# Autodesk Inventor assembly: 17-0028-0121
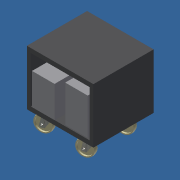
[picture p0: Inventor's stored thumbnail of the model, 180x180]
Saved by Autodesk Inventor 2019.1 (Build 231200000, 200)
## iProperties
Created: 2018-12-19
Part Number: 17-0028-0121
Document SubType Name: Assembly
Designer: D. Giesen
Author: D. Giesen
## Documents named in this file (4)
- D:\VaultLocalWorkingFolder\UvA_MT\Projects\2017\17-0028 Digital PID Loop\10_Assemblies\17-0028-0121.iam
- D:\VaultLocalWorkingFolder\UvA_MT\Projects\2017\17-0028 Digital PID Loop\20_3D-Models\17-0028-0036.iam
- D:\VaultLocalWorkingFolder\UvA_MT\Projects\2017\17-0028 Digital PID Loop\20_3D-Models\17-0028-0122.ipt
- D:\VaultLocalWorkingFolder\UvA_MT\Projects\2017\17-0028 Digital PID Loop\20_3D-Models\17-0028-0123.ipt
## Components (3 placed, 3 different names)
1. 17-0028-0036:1 [sub-assembly] — Mate:1, Mate:2
2. 17-0028-0122:1 — Mate:1
3. 17-0028-0123:1 — Mate:2
## Relationships (2: Mate 2)
- Mate:1: 17-0028-0036:1 ↔ 17-0028-0122:1
- Mate:2: 17-0028-0036:1 ↔ 17-0028-0123:1
